# Autodesk Inventor assembly: PivotMech2
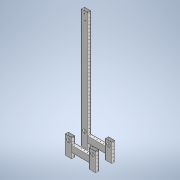
[picture p0: Inventor's stored thumbnail of the model, 180x180]
Saved by Autodesk Inventor 2022 (Build 260153000, 153)
## iProperties
Created: 2022-03-02
Part Number: PivotMech2
Document SubType Name: Assembly
Designer: tagaz
Author: tagaz
## Documents named in this file (4)
- C:\Users\tagaz\OneDrive\Documents\T3-Cad\CAD\2022 Parts\TelescopeElev\PivotMech\PivotMech2.iam
- C:\Users\tagaz\OneDrive\Documents\T3-Cad\CAD\2022 Parts\TelescopeElev\PivotMech\ElevatorPivotBar1.ipt
- C:\Users\tagaz\OneDrive\Documents\T3-Cad\CAD\2022 Parts\TelescopeElev\PivotMech\ElevatorPivotBar2.ipt
- C:\Users\tagaz\OneDrive\Documents\T3-Cad\CAD\2022 Parts\TelescopeElev\PivotMech\ElevatorPivotBar3.ipt
## Components (6 placed, 3 different names)
1. ElevatorPivotBar1:1 — Flush:1, Flush:2, Flush:3, Flush:4, Mate:6
2. ElevatorPivotBar1:6 — Flush:1, Flush:2, Flush:9, Mate:5, Flush:10, Mate:9
3. ElevatorPivotBar2:1 — Flush:3, Flush:4, Mate:6, Mate:9
4. ElevatorPivotBar1:3 — Mate:7
5. ElevatorPivotBar3:1 — Flush:9, Mate:5, Flush:10, Mate:8
6. ElevatorPivotBar2:2 — Mate:7, Mate:8
## Relationships (15: Flush 10, Mate 5)
- Flush:1: ElevatorPivotBar1:1 ↔ ElevatorPivotBar1:6
- Flush:2: ElevatorPivotBar1:1 ↔ ElevatorPivotBar1:6
- Flush:3: ElevatorPivotBar1:1 ↔ ElevatorPivotBar2:1
- Flush:4 (50.8 mm): ElevatorPivotBar1:1 ↔ ElevatorPivotBar2:1
- [Flush]: ElevatorPivotBar1:3 ↔ ElevatorPivotBar3:1
- [Flush]: ElevatorPivotBar1:3 ↔ ElevatorPivotBar3:1
- [Flush]: ElevatorPivotBar1:3 ↔ ElevatorPivotBar2:2
- [Flush] (50.8 mm): ElevatorPivotBar1:3 ↔ ElevatorPivotBar2:2
- Flush:9: ElevatorPivotBar1:6 ↔ ElevatorPivotBar3:1
- Mate:5 (101.6 mm): ElevatorPivotBar1:6 ↔ ElevatorPivotBar3:1
- Flush:10: ElevatorPivotBar1:6 ↔ ElevatorPivotBar3:1
- Mate:6: ElevatorPivotBar1:1 ↔ ElevatorPivotBar2:1
- Mate:7: ElevatorPivotBar1:3 ↔ ElevatorPivotBar2:2
- Mate:8: ElevatorPivotBar3:1 ↔ ElevatorPivotBar2:2
- Mate:9: ElevatorPivotBar1:6 ↔ ElevatorPivotBar2:1
## Named parameters: d6_d0 = 0 mm, d7_d1 = 0 mm, d8_d2 = 0 mm, d11_d5 = 50.8 mm
